# Autodesk Inventor assembly: Assembly
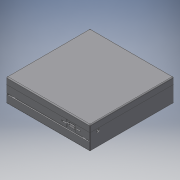
[picture p0: Inventor's stored thumbnail of the model, 180x180]
Saved by Autodesk Inventor 2018 (Build 220112000, 112)
## iProperties
Created: 2019-05-02
Part Number: Assembly
Document SubType Name: Assembly
Designer: thatg
Author: thatg
## Documents named in this file (3)
- C:\Users\thatg\Documents\Commodore Cube Project\Case\Assembly.iam
- C:\Users\thatg\Documents\Commodore Cube Project\Case\Tray.ipt
- C:\Users\thatg\Documents\Commodore Cube Project\Case\Dome.ipt
## Components (2 placed, 2 different names)
1. Tray:1 — Flush:1
2. Dome:1 — Flush:1
## Relationships (1: Flush 1)
- Flush:1: Tray:1 ↔ Dome:1
